# Autodesk Inventor assembly: MotorWheelAssembly
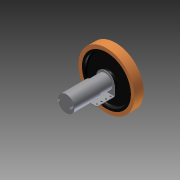
[picture p0: Inventor's stored thumbnail of the model, 180x180]
Saved by Autodesk Inventor 2012 (Build 160160000, 160)
## iProperties
Created: 2013-07-13
Part Number: MotorWheelAssembly
Document SubType Name: Assembly
Designer: joe_000
Author: joe_000
## Documents named in this file (6)
- C:\dev\telepresenceRobot\mechanical\MotorWheelAssembly.iam
- C:\dev\telepresenceRobot\mechanical\HD-BK-IG-MotorBracket.ipt
- C:\dev\telepresenceRobot\mechanical\IG32P-Motor.ipt
- C:\dev\telepresenceRobot\mechanical\T80P-494BO-HS6-Wheel.ipt
- C:\dev\telepresenceRobot\mechanical\T80H-SM61-WheelHub.ipt
- C:\Users\joe_000\Documents\Inventor\Content Center Files\R2012\en-US\ANSI B18.3.4M(1)\ANSI B18.3.4M - M3 x 0.5 x 5(2).ipt
## Components (6 placed, 5 different names)
1. HD-BK-IG-MotorBracket:1 — Insert:1, Insert:4, Insert:5
2. IG32P-Motor:1 — Insert:1, Insert:2, Mate:1
3. T80P-494BO-HS6-Wheel:1 — Insert:3, Angle:1
4. T80H-SM61-WheelHub:1 — Insert:2, Insert:3, Angle:1
5. Broached Hexagon Socket Button Head Cap Screw - Metric M3 x 0.5 x 5:1 — Insert:4, Mate:1
6. Broached Hexagon Socket Button Head Cap Screw - Metric M3 x 0.5 x 5:2 — Insert:5
## Relationships (7: Insert 5, Angle 1, Mate 1)
- Insert:1: HD-BK-IG-MotorBracket:1 ↔ IG32P-Motor:1
- Insert:2: IG32P-Motor:1 ↔ T80H-SM61-WheelHub:1
- Insert:3: T80P-494BO-HS6-Wheel:1 ↔ T80H-SM61-WheelHub:1
- Angle:1 (0 deg): T80P-494BO-HS6-Wheel:1 ↔ T80H-SM61-WheelHub:1
- Insert:4: HD-BK-IG-MotorBracket:1 ↔ Broached Hexagon Socket Button Head Cap Screw - Metric M3 x 0.5 x 5:1
- Mate:1: IG32P-Motor:1 ↔ Broached Hexagon Socket Button Head Cap Screw - Metric M3 x 0.5 x 5:1
- Insert:5: HD-BK-IG-MotorBracket:1 ↔ Broached Hexagon Socket Button Head Cap Screw - Metric M3 x 0.5 x 5:2
